# Autodesk Inventor assembly: RectangularHolderAssembled
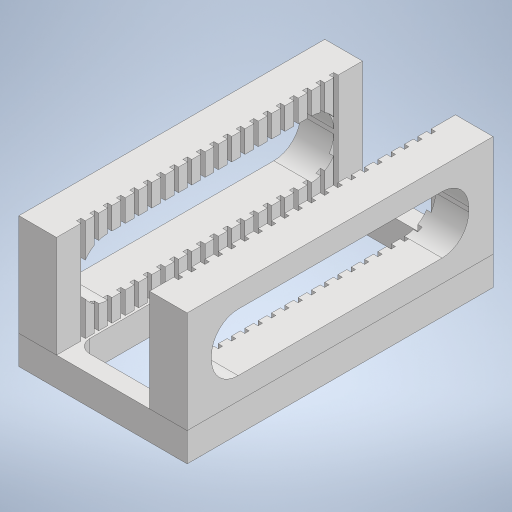
[picture p0: Inventor's stored thumbnail of the model, 512x512]
Saved by Autodesk Inventor 2024 (Build 280153000, 153)
## iProperties
Created: 2023-08-14
Part Number: RectangularHolderAssembled
Document SubType Name: Assembly
Designer: ewinden
Author: ewinden
## Documents named in this file (4)
- E:\Box Sync\Documents\Inventor\Schwartz Laqb\RectangularHolderAssembled.iam
- E:\Box Sync\Documents\Inventor\Schwartz Laqb\RectangularHolderFloor.ipt
- E:\Box Sync\Documents\Inventor\Schwartz Laqb\RectangularHolderWall.ipt
- E:\Box Sync\Documents\Inventor\Schwartz Laqb\PTFE Plastic Screw.ipt
## Components (7 placed, 3 different names)
1. RectangularHolderFloor:1 — Mate:1, Mate:2, Mate:3, Mate:4, Mate:5, Mate:6, Mate:7, Mate:8, Mate:9, Mate:10, Mate:11, Mate:12, Mate:13, Mate:14
2. RectangularHolderWall:1 — Mate:1, Mate:3, Mate:4
3. RectangularHolderWall:2 — Mate:2, Mate:5, Mate:6
4. PTFE Plastic Screw:1 — Mate:8, Mate:13
5. PTFE Plastic Screw:2 — Mate:7, Mate:14
6. PTFE Plastic Screw:3 — Mate:10, Mate:12
7. PTFE Plastic Screw:4 — Mate:9, Mate:11
## Relationships (14: Mate 14)
- Mate:1: RectangularHolderFloor:1 ↔ RectangularHolderWall:1
- Mate:2: RectangularHolderFloor:1 ↔ RectangularHolderWall:2
- Mate:3: RectangularHolderFloor:1 ↔ RectangularHolderWall:1
- Mate:4: RectangularHolderFloor:1 ↔ RectangularHolderWall:1
- Mate:5: RectangularHolderFloor:1 ↔ RectangularHolderWall:2
- Mate:6: RectangularHolderFloor:1 ↔ RectangularHolderWall:2
- Mate:7: RectangularHolderFloor:1 ↔ PTFE Plastic Screw:2
- Mate:8: RectangularHolderFloor:1 ↔ PTFE Plastic Screw:1
- Mate:9: RectangularHolderFloor:1 ↔ PTFE Plastic Screw:4
- Mate:10: RectangularHolderFloor:1 ↔ PTFE Plastic Screw:3
- Mate:11: RectangularHolderFloor:1 ↔ PTFE Plastic Screw:4
- Mate:12: RectangularHolderFloor:1 ↔ PTFE Plastic Screw:3
- Mate:13: RectangularHolderFloor:1 ↔ PTFE Plastic Screw:1
- Mate:14: RectangularHolderFloor:1 ↔ PTFE Plastic Screw:2
